# Autodesk Inventor assembly: ufo1.0
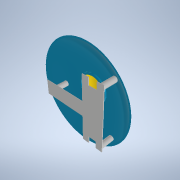
[picture p0: Inventor's stored thumbnail of the model, 180x180]
Saved by Autodesk Inventor 2020 (Build 240168000, 168)
## iProperties
Created: 2020-03-24
Part Number: ufo1.0
Document SubType Name: Assembly
Designer: magnu
Mass: 173.122 g
Surface Area: 1304.95 cm^2
Volume: 173.122 cm^3
Density: 1 g/cm^3
Author: magnu
## Documents named in this file (4)
- C:\Users\magnu\OneDrive\Documents\ufo1.0.iam
- C:\Users\magnu\OneDrive\Documents\bottenplatta.ipt
- C:\Users\magnu\OneDrive\Documents\topplock.ipt
- C:\Users\magnu\OneDrive\Documents\Part5.ipt
## Components (3 placed, 3 different names)
1. bottenplatta:1
2. topplock:1 — Insert:1
3. Part5:1 — Insert:1
## Relationships (1: Insert 1)
- Insert:1: topplock:1 ↔ Part5:1
